# Autodesk Inventor assembly: BG004_huenin20_23
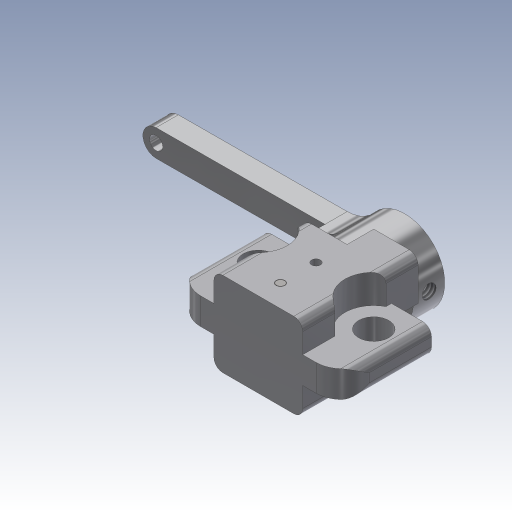
[picture p0: Inventor's stored thumbnail of the model, 512x512]
Saved by Autodesk Inventor 2023.3 (Build 273359000, 359)
## iProperties
Company: HTBLA Kaindorf
RuleStatus: InUse
Created: 2024-01-29
Part Number: BG004_huenin20_23
Project: Fiberprinter-Hotend
Material: Generisch
Description: SMN
Document SubType Name: Assembly
Designer: huenin20
Mass: 11.7206 g
Surface Area: 22.7428 cm^2
Volume: 1.81134 cm^3
Density: 6.47069 g/cm^3
AfterDocNew0: iProperties-Editor_aufrufen
Author: nicob
Keywords: 2023
## Documents named in this file (6)
- H:\Dokumente\Projects\Kop\Fiberprinter_Hotend\BG004_huenin20_23_Fiberprinter-Hotend_SMN.iam
- H:\Dokumente\Projects\Kop\Fiberprinter_Hotend\BT015_huenin20_23_Fiberprinter-Hotend_SMN_Gehäuse.ipt
- H:\Dokumente\Projects\Kop\Fiberprinter_Hotend\ISO 2338 - 3 m6 x 8.ipt
- H:\Dokumente\Projects\Kop\Fiberprinter_Hotend\DIN 179 - A 5 x 12.ipt
- H:\Dokumente\Projects\Kop\Fiberprinter_Hotend\Normteile\de-DE\ISO 2338(2)\ISO 2338 - 1 h8 x 4.ipt
- H:\Dokumente\Projects\Kop\Fiberprinter_Hotend\BT006_huenin20_23_Fiberprinter-Hotend_Schneidhebel.ipt
## Components (5 placed, 5 different names)
1. BT015_huenin20_23_Fiberprinter-Hotend_SMN_Gehäuse:1 — Winkel:2, Passend:11, Passend:12, Passend:13, Einfügen:1, Einfügen:3
2. DIN 179 - A 5 x 12:1 — Passend:12, Passend:13, Einfügen:2
3. ISO 2338 3 m6 x 8:1 — Passend:11, Einfügen:1, Winkel:3
4. ISO 2338 1 h8 x 4:1 — Einfügen:3
5. BT006_huenin20_23_Fiberprinter-Hotend_Schneidhebel:1 — Einfügen:2, Winkel:3
## Relationships (11: Mate 6, Insert 3, Angle 2)
- Passend:4 [Mate]
- Passend:5 [Mate]
- Passend:8 [Mate]
- Winkel:2 [Angle] (180 deg): BT015_huenin20_23_Fiberprinter-Hotend_SMN_Gehäuse:1
- Passend:11 [Mate]: BT015_huenin20_23_Fiberprinter-Hotend_SMN_Gehäuse:1 ↔ ISO 2338 3 m6 x 8:1
- Passend:12 [Mate]: BT015_huenin20_23_Fiberprinter-Hotend_SMN_Gehäuse:1 ↔ DIN 179 - A 5 x 12:1
- Passend:13 [Mate]: BT015_huenin20_23_Fiberprinter-Hotend_SMN_Gehäuse:1 ↔ DIN 179 - A 5 x 12:1
- Einfügen:1 [Insert]: BT015_huenin20_23_Fiberprinter-Hotend_SMN_Gehäuse:1 ↔ ISO 2338 3 m6 x 8:1
- Einfügen:2 [Insert]: DIN 179 - A 5 x 12:1 ↔ BT006_huenin20_23_Fiberprinter-Hotend_Schneidhebel:1
- Winkel:3 [Angle] (-90 deg): ISO 2338 3 m6 x 8:1 ↔ BT006_huenin20_23_Fiberprinter-Hotend_Schneidhebel:1
- Einfügen:3 [Insert]: BT015_huenin20_23_Fiberprinter-Hotend_SMN_Gehäuse:1 ↔ ISO 2338 1 h8 x 4:1
